# Autodesk Inventor assembly: Samling
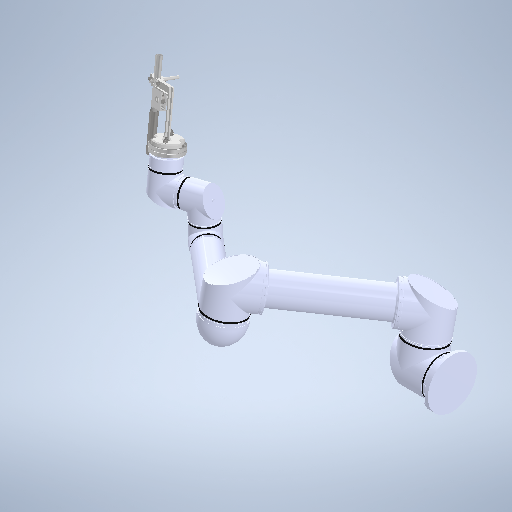
[picture p0: Inventor's stored thumbnail of the model, 512x512]
Saved by Autodesk Inventor 2025.1 (Build 291241000, 241)
## iProperties
Created: 2025-02-26
Part Number: Samling
Document SubType Name: Assembly
Designer: frede
Mass: 338.579 g
Surface Area: 412.497 cm^2
Volume: 65.2312 cm^3
Density: 5.19044 g/cm^3
Author: frede
## Documents named in this file (20)
- C:\Users\frede\OneDrive\Skole\SDU\2. Semester\Semesterprojekt\3D model\Samling.iam
- C:\Users\frede\OneDrive\Skole\SDU\2. Semester\Semesterprojekt\3D model\Rør.ipt
- C:\Users\frede\OneDrive\Skole\SDU\2. Semester\Semesterprojekt\3D model\Stempel.ipt
- C:\Users\frede\OneDrive\Skole\SDU\2. Semester\Semesterprojekt\3D model\tandhjul.ipt
- C:\Users\frede\OneDrive\Skole\SDU\2. Semester\Semesterprojekt\3D model\Samling\Design Accelerator\Spur Gears3.iam
- C:\Users\frede\OneDrive\Skole\SDU\2. Semester\Semesterprojekt\3D model\Fjeder_Hus.ipt
- C:\Users\frede\OneDrive\Skole\SDU\2. Semester\Semesterprojekt\3D model\Ø10-Ø8Prop.ipt
- C:\Users\frede\OneDrive\Skole\SDU\2. Semester\Semesterprojekt\3D model\HandCrank.ipt
- C:\Users\frede\OneDrive\Skole\SDU\2. Semester\Semesterprojekt\3D model\STL\RobotarmHolder.ipt
- C:\Users\frede\OneDrive\Skole\SDU\2. Semester\Semesterprojekt\3D model\UR5 Gripper Interface plate.ipt
- C:\Users\frede\OneDrive\Skole\SDU\2. Semester\Semesterprojekt\3D model\UR5\24105_Support\24105_Support\24105_Support.iam
- C:\Users\frede\OneDrive\Dokumenter\Inventor\Content Center Files\R2025\en-US\ISO 4762(2)\ISO 4762 - M6 x 10ISO.ipt
- C:\Users\frede\OneDrive\Skole\SDU\2. Semester\Semesterprojekt\3D model\UR5 Gripper Interface 2 robot plate.ipt
- C:\Users\frede\OneDrive\Dokumenter\Inventor\Content Center Files\R2025\en-US\ISO 4762(2)\ISO 4762 - M6 x 25ISO.ipt
- C:\Users\frede\OneDrive\Dokumenter\Inventor\Content Center Files\R2025\en-US\DIN 125-1  B\DIN 125-1 - B 6,4.ipt
- C:\Users\frede\OneDrive\Dokumenter\Inventor\Content Center Files\R2025\en-US\ISO 4032(2)\ISO 4032 - M6 - ISO.ipt
- C:\Users\frede\OneDrive\Skole\SDU\2. Semester\Semesterprojekt\3D model\STL\RobotarmHolderSpaende.ipt
- C:\Users\frede\OneDrive\Dokumenter\Inventor\Content Center Files\R2025\en-US\DIN 128\DIN 128 - A5.ipt
- C:\Users\frede\OneDrive\Dokumenter\Inventor\Content Center Files\R2025\en-US\ISO 4762(2)\ISO 4762 - M5 x 16ISO.ipt
- C:\Users\frede\OneDrive\Dokumenter\Inventor\Content Center Files\R2025\en-US\DIN EN ISO 4032\DIN EN ISO 4032 - M5.ipt
## Components (33 placed, 19 different names)
1. 24105_Support:1 [sub-assembly] — Rotational:6, Mate:4
2. Rør:1 — Mate:1, Rotational:2, Rotational:3, Cylindrical:1, Angle:3, Mate:2, Mate:3, Angle:4, Mate:7, Mate:13
3. Stempel:1 — Rotation/Translation:1, Mate:1, Angle:3
4. tandhjul:1 — Rotation/Translation:1, Angle:2, Rotational:4, Rotational:5
5. Spur Gears:1 [sub-assembly]
6. Fjeder_Hus:1 — Cylindrical:1, Mate:7
7. Ø10-Ø8Prop:1 — Rotational:2
8. Ø10-Ø8Prop:2 — Rotational:3, Rotational:5
9. HandCrank:1 — Angle:2, Rotational:4
10. RobotarmHolder:1 — Mate:2, Mate:3, Angle:4, Mate:8, Mate:9, Mate:10, Mate:11, Mate:12, Insert:9, Insert:10, Insert:15, Insert:16
11. UR5 Gripper Interface plate:1 — Rotational:6, Mate:4, Insert:1, Insert:2, Insert:3, Insert:4, Rotational:7, Mate:5
12. ISO 4762 M6 x 10:1 — Insert:1
13. ISO 4762 M6 x 10:2 — Insert:2
14. ISO 4762 M6 x 10:3 — Insert:3
15. ISO 4762 M6 x 10:4 — Insert:4
16. UR5 Gripper Interface 2 robot plate:1 — Rotational:7, Mate:5, Insert:5, Insert:6, Mate:8, Mate:9, Mate:10, Mate:11, Mate:12, Insert:7, Insert:8
17. ISO 4762 M6 x 10:5 — Insert:5
18. ISO 4762 M6 x 10:6 — Insert:6
19. ISO 4762 M6 x 25:1 — Insert:7
20. ISO 4762 M6 x 25:2 — Insert:8
21. DIN 125-1 B B 6,4:1 — Insert:9, Insert:11
22. DIN 125-1 B B 6,4:2 — Insert:10, Insert:12
23. ISO 4032 M6:1 — Insert:11
24. ISO 4032 M6:2 — Insert:12
25. RobotarmHolderSpaende:1 — Mate:13, Insert:13, Insert:14
26. DIN 128 A5:1 — Insert:13, Insert:17
27. DIN 128 A5:2 — Insert:14, Insert:18
28. DIN 128 A5:3 — Insert:15, Insert:20
29. DIN 128 A5:4 — Insert:16, Insert:19
30. ISO 4762 M5 x 16:1 — Insert:17
31. ISO 4762 M5 x 16:2 — Insert:18
32. DIN EN ISO 4032 M5:1 — Insert:19
33. DIN EN ISO 4032 M5:2 — Insert:20
## Relationships (43: Insert 20, Mate 12, RevoluteJoint 6, Angle 3, RelateRotateTranslate 1, CylindricalJoint 1)
- Rotation/Translation:1 [RelateRotateTranslate] (91.634 mm): Stempel:1 ↔ tandhjul:1
- Mate:1: Rør:1 ↔ Stempel:1
- Rotational:2 [RevoluteJoint]: Rør:1 ↔ Ø10-Ø8Prop:1
- Rotational:3 [RevoluteJoint]: Rør:1 ↔ Ø10-Ø8Prop:2
- Cylindrical:1: Rør:1 ↔ Fjeder_Hus:1
- Angle:2 (180 deg): tandhjul:1 ↔ HandCrank:1
- Rotational:4 [RevoluteJoint]: tandhjul:1 ↔ HandCrank:1
- Angle:3 (0 deg): Rør:1 ↔ Stempel:1
- Rotational:5 [RevoluteJoint]: tandhjul:1 ↔ Ø10-Ø8Prop:2
- Mate:2: Rør:1 ↔ RobotarmHolder:1
- Mate:3 (3.5 mm): Rør:1 ↔ RobotarmHolder:1
- Rotational:6 [RevoluteJoint]: 24105_Support:1 ↔ UR5 Gripper Interface plate:1
- Mate:4: 24105_Support:1 ↔ UR5 Gripper Interface plate:1
- Insert:1: UR5 Gripper Interface plate:1 ↔ ISO 4762 M6 x 10:1
- Insert:2: UR5 Gripper Interface plate:1 ↔ ISO 4762 M6 x 10:2
- Insert:3: UR5 Gripper Interface plate:1 ↔ ISO 4762 M6 x 10:3
- Insert:4: UR5 Gripper Interface plate:1 ↔ ISO 4762 M6 x 10:4
- Rotational:7 [RevoluteJoint]: UR5 Gripper Interface plate:1 ↔ UR5 Gripper Interface 2 robot plate:1
- Mate:5: UR5 Gripper Interface plate:1 ↔ UR5 Gripper Interface 2 robot plate:1
- Insert:5: UR5 Gripper Interface 2 robot plate:1 ↔ ISO 4762 M6 x 10:5
- Insert:6: UR5 Gripper Interface 2 robot plate:1 ↔ ISO 4762 M6 x 10:6
- Angle:4 (180 deg): Rør:1 ↔ RobotarmHolder:1
- Mate:7 (10 mm): Rør:1 ↔ Fjeder_Hus:1
- Mate:8: RobotarmHolder:1 ↔ UR5 Gripper Interface 2 robot plate:1
- Mate:9: RobotarmHolder:1 ↔ UR5 Gripper Interface 2 robot plate:1
- Mate:10: RobotarmHolder:1 ↔ UR5 Gripper Interface 2 robot plate:1
- Mate:11: RobotarmHolder:1 ↔ UR5 Gripper Interface 2 robot plate:1
- Mate:12: RobotarmHolder:1 ↔ UR5 Gripper Interface 2 robot plate:1
- Insert:7: UR5 Gripper Interface 2 robot plate:1 ↔ ISO 4762 M6 x 25:1
- Insert:8: UR5 Gripper Interface 2 robot plate:1 ↔ ISO 4762 M6 x 25:2
- Insert:9: RobotarmHolder:1 ↔ DIN 125-1 B B 6,4:1
- Insert:10: RobotarmHolder:1 ↔ DIN 125-1 B B 6,4:2
- Insert:11: DIN 125-1 B B 6,4:1 ↔ ISO 4032 M6:1
- Insert:12: DIN 125-1 B B 6,4:2 ↔ ISO 4032 M6:2
- Mate:13: Rør:1 ↔ RobotarmHolderSpaende:1
- Insert:13: RobotarmHolderSpaende:1 ↔ DIN 128 A5:1
- Insert:14: RobotarmHolderSpaende:1 ↔ DIN 128 A5:2
- Insert:15: RobotarmHolder:1 ↔ DIN 128 A5:3
- Insert:16: RobotarmHolder:1 ↔ DIN 128 A5:4
- Insert:17: DIN 128 A5:1 ↔ ISO 4762 M5 x 16:1
- Insert:18: DIN 128 A5:2 ↔ ISO 4762 M5 x 16:2
- Insert:19: DIN 128 A5:4 ↔ DIN EN ISO 4032 M5:1
- Insert:20: DIN 128 A5:3 ↔ DIN EN ISO 4032 M5:2
